# Autodesk Inventor assembly: Right Assembly
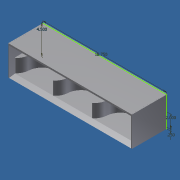
[picture p0: Inventor's stored thumbnail of the model, 180x180]
Saved by Autodesk Inventor 2012 (Build 160160000, 160)
## iProperties
Created: 2012-02-03
Part Number: Right Assembly
Document SubType Name: Assembly
Designer: Allison Garza
Author: Allison Garza
## Documents named in this file (6)
- C:\Users\Allison Garza\Documents\Rice Spring 2012\MRSL\Right Assembly.iam
- C:\Users\Allison Garza\Documents\Rice Spring 2012\circuit board.ipt
- C:\Users\Allison Garza\Documents\Rice Spring 2012\swirvy.ipt
- C:\Users\Allison Garza\Documents\Rice Spring 2012\MRSL\side panel.ipt
- C:\Users\Allison Garza\Documents\Rice Spring 2012\MRSL\top and bottom panel normal.ipt
- C:\Users\Allison Garza\Documents\Rice Spring 2012\MRSL\bottom panel.ipt
## Components (6 placed, 5 different names)
1. circuit board:1 — Mate:1, Mate:2, Flush:1, Mate:4, Flush:2, Mate:5, Flush:3, Flush:4, Mate:6, Mate:8
2. swirvy:1 — Mate:1, Mate:2, Flush:1, Mate:3
3. side panel:1 — Mate:3, Mate:4, Flush:2, Mate:7, Flush:5
4. side panel:2 — Mate:5, Flush:3, Flush:4, Mate:9, Flush:6
5. top and bottom panel normal:1 — Mate:6, Mate:7, Flush:5
6. bottom panel:1 — Mate:8, Mate:9, Flush:6
## Relationships (15: Mate 9, Flush 6)
- Mate:1: circuit board:1 ↔ swirvy:1
- Mate:2: circuit board:1 ↔ swirvy:1
- Flush:1 (-3.175 mm): circuit board:1 ↔ swirvy:1
- Mate:3: swirvy:1 ↔ side panel:1
- Mate:4: circuit board:1 ↔ side panel:1
- Flush:2: circuit board:1 ↔ side panel:1
- Mate:5: circuit board:1 ↔ side panel:2
- Flush:3: circuit board:1 ↔ side panel:2
- Flush:4: circuit board:1 ↔ side panel:2
- Mate:6: circuit board:1 ↔ top and bottom panel normal:1
- Mate:7: side panel:1 ↔ top and bottom panel normal:1
- Flush:5: side panel:1 ↔ top and bottom panel normal:1
- Mate:8: circuit board:1 ↔ bottom panel:1
- Mate:9: side panel:2 ↔ bottom panel:1
- Flush:6: side panel:2 ↔ bottom panel:1
